# Autodesk Inventor assembly: Hold_18650-2p_smd
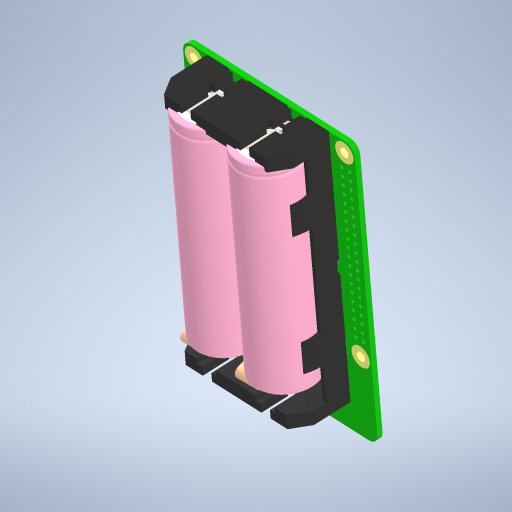
[picture p0: Inventor's stored thumbnail of the model, 512x512]
Saved by Autodesk Inventor 2023 (Build 270158000, 158)
## iProperties
Company: UNSPECIFIED
Created: 1900-01-01
Part Number: Hold_18650-2p_smd
Description: STEP AP214
Document SubType Name: Assembly
Designer: tdal0
Title: Hold_18650-2p_smd
Author: UNSPECIFIED
Revision Number: ANYUNSPECIFIED
Sending System: C3D Toolkit
Preprocessor: C3D Converter
## Documents named in this file (5)
- C:\4805\front panel parts\Hold_18650-2p_smd.iam
- C:\4805\front panel parts\Hold_18650_Con_smd.ipt
- C:\4805\front panel parts\Hold_18650-2p_smd.ipt
- C:\4805\front panel parts\18650 v4.ipt
- C:\4805\front panel parts\Raspberry Pi 4 Model B.ipt
## Components (6 placed, 3 different names)
1. ANY — Mate:4
2. ANY:2 — Mate:3, Mate:5, Mate:7, Flush:1
3. ANY:4 — Mate:6
4. 18650 v4:1 — Mate:3, Mate:4
5. 18650 v4:2 — Mate:5, Mate:6
6. Raspberry Pi 4 Model B:1 — Mate:7, Flush:1
## Relationships (6: Mate 5, Flush 1)
- Mate:3: ANY:2 ↔ 18650 v4:1
- Mate:4: ANY ↔ 18650 v4:1
- Mate:5: ANY:2 ↔ 18650 v4:2
- Mate:6: ANY:4 ↔ 18650 v4:2
- Mate:7: ANY:2 ↔ Raspberry Pi 4 Model B:1
- Flush:1: ANY:2 ↔ Raspberry Pi 4 Model B:1
